# Autodesk Inventor assembly: Alternative Pump Assembley
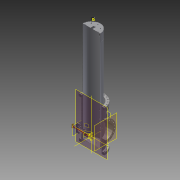
[picture p0: Inventor's stored thumbnail of the model, 180x180]
Saved by Autodesk Inventor 2015 (Build 190159000, 159)
## iProperties
Created: 2014-05-21
Part Number: Alternative Pump Assembley
Document SubType Name: Assembly
Designer: jad211
Author: jad211
## Documents named in this file (12)
- C:\CADFiles\EDM Machine\EDM New Pumping Region\Alternative Pump Assembley.iam
- C:\CADFiles\EDM Machine\EDM New Pumping Region\NewHorn.ipt
- C:\CADFiles\EDM Machine\EDM Beamline\Chamber parts\hudson chamber actual size.ipt
- C:\CADFiles\EDM Machine\EDM Inner Shield\Inner Shield.iam
- C:\CADFiles\EDM Machine\EDM New Pumping Region\bendy bit.ipt
- C:\CADFiles\EDM Machine\EDM New Pumping Region\ringLoop.ipt
- C:\CADFiles\EDM Machine\EDM New Pumping Region\table.ipt
- C:\CADFiles\EDM Machine\EDM New Pumping Region\3-38WithHoles.ipt
- C:\CADFiles\EDM Machine\EDM New Pumping Region\WG18FLANGE.ipt
- C:\CADFiles\EDM Machine\EDM New Pumping Region\WG18FLANGECutDown.ipt
- C:\CADFiles\Generic vacuum components\SMA feedthrough 338\F0275X0501P_3.ipt
- C:\CADFiles\EDM Machine\EDM New Pumping Region\loop holder.ipt
## Components (17 placed, 11 different names)
1. NewHorn:1 — Angle:1, Mate:5, Angle:2, Mate:6, Mate:7, Mate:8, Angle:3, Mate:13, Mate:21, Mate:22, Flush:8, Angle:4, Mate:29, Flush:11, Mate:30, Angle:5
2. hudson chamber actual size:1 — Mate:1, Mate:2, Mate:3, Mate:16
3. Inner Shield:1 [sub-assembly] — Mate:3, Mate:4, Flush:1, Mate:9, Mate:10
4. bendy bit:1 — Mate:6, Mate:7, Mate:14, Mate:15, Flush:5, Mate:17, Mate:18, Mate:20
5. ringLoop:1 — Mate:26, Mate:27
6. table:1 — Flush:1, Mate:9, Mate:10
7. ringLoop:2 — Mate:24, Mate:25, Flush:6
8. 3-38WithHoles:1 — Mate:14, Mate:15, Mate:16, Flush:5, Insert:1, Insert:2, Insert:3, Insert:4
9. WG18FLANGE:1 — Mate:17, Mate:18
10. WG18FLANGECutDown:1 — Mate:20, Mate:21, Mate:23
11. WG18FLANGECutDown:2 — Mate:22, Mate:23
12. F0275X0501P_3:1 — Insert:4
13. F0275X0501P_3:2 — Insert:3
14. F0275X0501P_3:3 — Insert:2
15. F0275X0501P_3:4 — Insert:1
16. loop holder:1 — Mate:28, Angle:4, Flush:10, Mate:29
17. loop holder:2 — Flush:11, Mate:30, Angle:5
## Relationships (44: Mate 28, Flush 7, Angle 5, Insert 4)
- Mate:1: hudson chamber actual size:1
- Mate:2: hudson chamber actual size:1
- Mate:3: hudson chamber actual size:1 ↔ Inner Shield:1
- Mate:4: Inner Shield:1
- Angle:1 (90 deg): NewHorn:1
- Mate:5: NewHorn:1
- Angle:2 (195 deg): NewHorn:1
- Mate:6: NewHorn:1 ↔ bendy bit:1
- Mate:7: NewHorn:1 ↔ bendy bit:1
- Mate:8: NewHorn:1
- Flush:1: Inner Shield:1 ↔ table:1
- Mate:9: Inner Shield:1 ↔ table:1
- Mate:10: Inner Shield:1 ↔ table:1
- Mate:12
- Angle:3 (0 deg): NewHorn:1
- Mate:13 (13 mm): NewHorn:1
- Mate:14: bendy bit:1 ↔ 3-38WithHoles:1
- Mate:15: bendy bit:1 ↔ 3-38WithHoles:1
- Mate:16: hudson chamber actual size:1 ↔ 3-38WithHoles:1
- Flush:5 (-38.838 mm): bendy bit:1 ↔ 3-38WithHoles:1
- Mate:17: bendy bit:1 ↔ WG18FLANGE:1
- Mate:18: bendy bit:1 ↔ WG18FLANGE:1
- Mate:20: bendy bit:1 ↔ WG18FLANGECutDown:1
- Mate:21: NewHorn:1 ↔ WG18FLANGECutDown:1
- Mate:22: NewHorn:1 ↔ WG18FLANGECutDown:2
- Mate:23: WG18FLANGECutDown:1 ↔ WG18FLANGECutDown:2
- Insert:1: 3-38WithHoles:1 ↔ F0275X0501P_3:4
- Insert:2: 3-38WithHoles:1 ↔ F0275X0501P_3:3
- Insert:3: 3-38WithHoles:1 ↔ F0275X0501P_3:2
- Insert:4: 3-38WithHoles:1 ↔ F0275X0501P_3:1
- Mate:24: ringLoop:2
- Mate:25: ringLoop:2
- Flush:6 (8 mm): ringLoop:2
- Mate:26: ringLoop:1
- Mate:27 (8 mm): ringLoop:1
- Flush:8: NewHorn:1
- Flush:9
- Mate:28 (-16 mm): loop holder:1
- Angle:4 (180 deg): NewHorn:1 ↔ loop holder:1
- Flush:10: loop holder:1
- Mate:29: NewHorn:1 ↔ loop holder:1
- Flush:11: NewHorn:1 ↔ loop holder:2
- Mate:30: NewHorn:1 ↔ loop holder:2
- Angle:5 (0 deg): NewHorn:1 ↔ loop holder:2
